# Autodesk Inventor assembly: Chassis, Wheels, and Drive Train Assembly
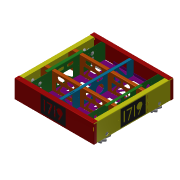
[picture p0: Inventor's stored thumbnail of the model, 180x180]
Saved by Autodesk Inventor 2015 (Build 190159000, 159)
## iProperties
Created: 2015-01-24
Part Number: Chassis, Wheels, and Drive Train Assembly
Document SubType Name: Assembly
Designer: Peter
Author: Peter
## Documents named in this file (4)
- T:\FILES\FIRST-Team-1719-CAD-Team\2015 Robot CAD\Chassis, Wheels, and Drive Train\Chassis, Wheels, and Drive Train Assembly.iam
- T:\FILES\FIRST-Team-1719-CAD-Team\2015 Robot CAD\Chassis, Wheels, and Drive Train\Chassis\Full chassis-3.iam
- T:\FILES\FIRST-Team-1719-CAD-Team\2015 Robot CAD\Number Plate\Number Plate.ipt
- T:\FILES\FIRST-Team-1719-CAD-Team\2015 Robot CAD\Chassis, Wheels, and Drive Train\Mechanum Wheel\Chassis - Wheel.iam
## Components (9 placed, 3 different names)
1. Full chassis-3:1 [sub-assembly] — Mate:1, Mate:2, Mate:3, Mate:4, Flush:1, Flush:2, Flush:3, Flush:4, Flush:5, Flush:6, Flush:7, Flush:8, Mate:5, Mate:6, Mate:7, Mate:8, Flush:9, Flush:10, Flush:11, Flush:12
2. Number Plate:1 — Mate:3, Flush:1, Flush:7
3. Number Plate:2 — Mate:4, Flush:2, Flush:6
4. Number Plate:3 — Mate:1, Flush:3, Flush:5
5. Number Plate:4 — Mate:2, Flush:4, Flush:8
6. Chassis - Wheel:1 [sub-assembly] — Mate:7, Flush:10
7. Chassis - Wheel:2 [sub-assembly] — Mate:8, Flush:9
8. Chassis - Wheel:3 [sub-assembly] — Mate:5, Flush:12
9. Chassis - Wheel:4 [sub-assembly] — Mate:6, Flush:11
## Relationships (20: Flush 12, Mate 8)
- Mate:1: Full chassis-3:1 ↔ Number Plate:3
- Mate:2: Full chassis-3:1 ↔ Number Plate:4
- Mate:3: Full chassis-3:1 ↔ Number Plate:1
- Mate:4: Full chassis-3:1 ↔ Number Plate:2
- Flush:1 (6.35 mm): Full chassis-3:1 ↔ Number Plate:1
- Flush:2 (6.35 mm): Full chassis-3:1 ↔ Number Plate:2
- Flush:3 (6.35 mm): Full chassis-3:1 ↔ Number Plate:3
- Flush:4 (6.35 mm): Full chassis-3:1 ↔ Number Plate:4
- Flush:5 (234.95 mm): Full chassis-3:1 ↔ Number Plate:3
- Flush:6 (234.95 mm): Full chassis-3:1 ↔ Number Plate:2
- Flush:7 (234.95 mm): Full chassis-3:1 ↔ Number Plate:1
- Flush:8 (234.95 mm): Full chassis-3:1 ↔ Number Plate:4
- Mate:5: Full chassis-3:1 ↔ Chassis - Wheel:3
- Mate:6: Full chassis-3:1 ↔ Chassis - Wheel:4
- Mate:7: Full chassis-3:1 ↔ Chassis - Wheel:1
- Mate:8: Full chassis-3:1 ↔ Chassis - Wheel:2
- Flush:9: Full chassis-3:1 ↔ Chassis - Wheel:2
- Flush:10: Full chassis-3:1 ↔ Chassis - Wheel:1
- Flush:11: Full chassis-3:1 ↔ Chassis - Wheel:4
- Flush:12: Full chassis-3:1 ↔ Chassis - Wheel:3
